# Autodesk Inventor assembly: узел бутылки
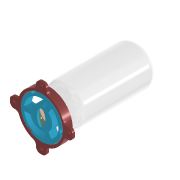
[picture p0: Inventor's stored thumbnail of the model, 180x180]
Saved by Autodesk Inventor 2022 (Build 260153000, 153)
## iProperties
Created: 2025-02-10
Part Number: узел бутылки
Document SubType Name: Assembly
Designer: User
Author: User
## Documents named in this file (4)
- E:\ВСЕ ДЕТАЛИ\узел бутылки.iam
- E:\ВСЕ ДЕТАЛИ\Основание бутылки.ipt
- E:\ВСЕ ДЕТАЛИ\переходник бутылки.ipt
- E:\shoter4\Бутылка_2.ipt
## Components (3 placed, 3 different names)
1. Основание бутылки:1 — Заподлицо:1, Совмещение:1
2. переходник бутылки:1 — Вставка:1, Заподлицо:1, Совмещение:1
3. Бутылка_2:1 — Вставка:1
## Relationships (3: Insert 1, Flush 1, Mate 1)
- Вставка:1 [Insert]: переходник бутылки:1 ↔ Бутылка_2:1
- Заподлицо:1 [Flush]: Основание бутылки:1 ↔ переходник бутылки:1
- Совмещение:1 [Mate]: Основание бутылки:1 ↔ переходник бутылки:1
